# Autodesk Inventor assembly: Lady Brown
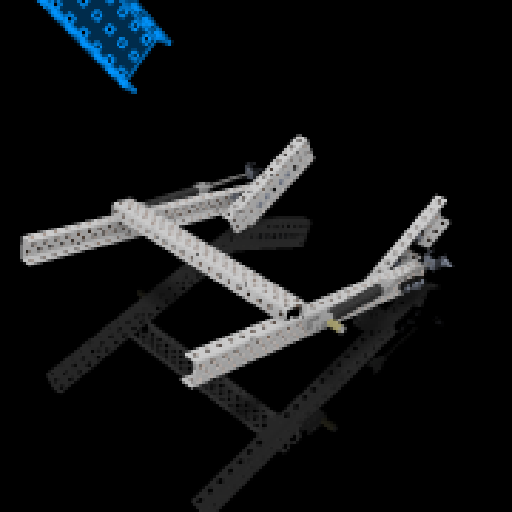
[picture p0: Inventor's stored thumbnail of the model, 512x512]
Saved by Autodesk Inventor 2025 (Build 290162000, 162)
## iProperties
Created: 2024-12-19
Part Number: Lady Brown
Document SubType Name: Assembly
Designer: Juan
Author: Juan
## Documents named in this file (20)
- C:\Users\Juan\Documents\GitHub\ATUM-VRC-High-Stakes-CAD\Robot\Subassemblies\Lady Brown.iam
- C:\Users\Juan\Documents\GitHub\ATUM-VRC-High-Stakes-CAD\VEX-CAD-Inventor\Structure\C Channel\Aluminum 1x2x1\Alu C 1x2x1x25.ipt
- C:\Users\Juan\Documents\GitHub\ATUM-VRC-High-Stakes-CAD\VEX-CAD-Inventor\Structure\C Channel\Aluminum 1x2x1\Alu C 1x2x1x19.ipt
- C:\Users\Juan\Documents\GitHub\ATUM-VRC-High-Stakes-CAD\VEX-CAD-Inventor\Motion\Spacers\Spacer Nylon .375 OD\NSpacer .375 OD x .500.ipt
- C:\Users\Juan\Documents\GitHub\ATUM-VRC-High-Stakes-CAD\VEX-CAD-Inventor\Motion\Spacers\Spacer Nylon .375 OD.ipt
- C:\Users\Juan\Documents\GitHub\ATUM-VRC-High-Stakes-CAD\VEX-CAD-Inventor\Motion\Pneumatics\Reference Parts\Pistons\Double Acting Piston Body.ipt
- C:\Users\Juan\Documents\GitHub\ATUM-VRC-High-Stakes-CAD\VEX-CAD-Inventor\Motion\Pneumatics\Reference Parts\Pistons\Double Acting Piston Rod.ipt
- C:\Users\Juan\Documents\GitHub\ATUM-VRC-High-Stakes-CAD\VEX-CAD-Inventor\Motion\Pneumatics\Legacy - SMC Pneumatics\Fitting for Cylinders.ipt
- C:\Users\Juan\Documents\GitHub\ATUM-VRC-High-Stakes-CAD\VEX-CAD-Inventor\Motion\Shaft LS\Bearing Flat.ipt
- C:\Users\Juan\Documents\GitHub\ATUM-VRC-High-Stakes-CAD\VEX-CAD-Inventor\Structure\Hardware\Screw Steel - Star\SScrew Star Smooth .500.ipt
- C:\Users\Juan\Documents\GitHub\ATUM-VRC-High-Stakes-CAD\VEX-CAD-Inventor\Structure\Hardware\Screw Steel - Star.ipt
- C:\Users\Juan\Documents\GitHub\ATUM-VRC-High-Stakes-CAD\VEX-CAD-Inventor\Structure\C Channel\Aluminum 1x3x1\Alu C 1x3x1x11.ipt
- C:\Users\Juan\Documents\GitHub\ATUM-VRC-High-Stakes-CAD\VEX-CAD-Inventor\Motion\1-Post Bearing Flat Hex Retainer.ipt
- C:\Users\Juan\Documents\GitHub\ATUM-VRC-High-Stakes-CAD\VEX-CAD-Inventor\Motion\Pneumatics\Legacy - SMC Pneumatics\Cylinder Mount.ipt
- C:\Users\Juan\Documents\GitHub\ATUM-VRC-High-Stakes-CAD\VEX-CAD-Inventor\Motion\Spacers\Spacer Nylon .375 OD\NSpacer .375 OD x .375.ipt
- C:\Users\Juan\Documents\GitHub\ATUM-VRC-High-Stakes-CAD\VEX-CAD-Inventor\Structure\Hardware\Screw Steel - Star\SScrew Star Smooth 2.250.ipt
- C:\Users\Juan\Documents\GitHub\ATUM-VRC-High-Stakes-CAD\VEX-CAD-Inventor\Structure\Hardware\Nut Nylock.ipt
- C:\Users\Juan\Documents\GitHub\ATUM-VRC-High-Stakes-CAD\VEX-CAD-Inventor\Structure\Hardware\Screw Steel - Star\SScrew Star Smooth 1.750.ipt
- C:\Users\Juan\Documents\GitHub\ATUM-VRC-High-Stakes-CAD\VEX-CAD-Inventor\Structure\Hardware\Nut Thin Nylock.ipt
- C:\Users\Juan\Documents\GitHub\ATUM-VRC-High-Stakes-CAD\VEX-CAD-Inventor\Structure\Hardware\Screw Steel - Star\SScrew Star Smooth .375.ipt
## Components (57 placed, 17 different names)
1. Alu C 1x2x1x25:1
2. Alu C 1x2x1x25:2
3. Alu C 1x2x1x19:1
4. NSpacer .375 OD x .500:1
5. NSpacer .375 OD x .500:2
6. Double Acting Piston Body:1
7. Double Acting Piston Rod:1
8. Fitting for Cylinders:1
9. Bearing Flat:1
10. SScrew Star Smooth .500:1
11. SScrew Star Smooth .500:2
12. Alu C 1x3x1x11:1
13. 1-Post Bearing Flat Hex Retainer:1
14. 1-Post Bearing Flat Hex Retainer:2
15. Cylinder Mount:1
16. NSpacer .375 OD x .375:3
17. NSpacer .375 OD x .500:4
18. NSpacer .375 OD x .375:5
19. NSpacer .375 OD x .500:6
20. SScrew Star Smooth 2.250:3
21. Nut Nylock:1
22. SScrew Star Smooth 1.750:4
23. Nut Thin Nylock:1
24. Nut Nylock:2
25. SScrew Star Smooth .375:5
26. SScrew Star Smooth .375:6
27. Nut Nylock:3
28. Double Acting Piston Body:2
29. Double Acting Piston Rod:2
30. NSpacer .375 OD x .500:13
31. NSpacer .375 OD x .375:14
32. Nut Thin Nylock:4
33. Nut Thin Nylock:3
34. Nut Thin Nylock:6
35. Nut Thin Nylock:5
36. SScrew Star Smooth 2.250:12
37. NSpacer .375 OD x .500:12
38. Fitting for Cylinders:2
39. Bearing Flat:2
40. SScrew Star Smooth .500:7
41. SScrew Star Smooth .500:8
42. Alu C 1x3x1x11:2
43. NSpacer .375 OD x .500:10
44. NSpacer .375 OD x .500:11
45. Cylinder Mount:2
46. NSpacer .375 OD x .500:7
47. Nut Nylock:4
48. Nut Thin Nylock:2
49. Nut Nylock:5
50. SScrew Star Smooth .375:9
51. SScrew Star Smooth .375:10
52. Nut Nylock:6
53. 1-Post Bearing Flat Hex Retainer:3
54. 1-Post Bearing Flat Hex Retainer:4
55. SScrew Star Smooth 1.750:11
56. NSpacer .375 OD x .500:8
57. NSpacer .375 OD x .375:9
## Relationships (93: Mate 58, WeldJoint 32, CylindricalJoint 2, RevoluteJoint 1)
- [Mate]: Alu C 1x2x1x25:1 ↔ Alu C 1x2x1x19:1
- [Mate]: Alu C 1x2x1x25:1 ↔ Alu C 1x2x1x19:1
- [Mate]: Alu C 1x2x1x25:2 ↔ Alu C 1x2x1x19:1
- [Mate]: Alu C 1x2x1x25:2 ↔ Alu C 1x2x1x19:1
- [Mate]: Alu C 1x2x1x19:1 ↔ NSpacer .375 OD x .500:1
- [Mate]: Alu C 1x2x1x19:1 ↔ NSpacer .375 OD x .500:2
- [Mate]: Alu C 1x2x1x19:1 ↔ NSpacer .375 OD x .500:2
- [Mate]: Alu C 1x2x1x19:1 ↔ NSpacer .375 OD x .500:1
- [Mate]: Alu C 1x2x1x25:1 ↔ NSpacer .375 OD x .500:2
- [Mate]: Double Acting Piston Body:1 ↔ Double Acting Piston Rod:1
- [CylindricalJoint]: Double Acting Piston Body:1 ↔ Double Acting Piston Rod:1
- [Mate]: Double Acting Piston Body:1 ↔ Fitting for Cylinders:1
- [Mate]: Double Acting Piston Body:1 ↔ Fitting for Cylinders:1
- [Mate]: Alu C 1x2x1x25:1 ↔ Bearing Flat:1
- [Mate]: Alu C 1x2x1x25:1 ↔ Bearing Flat:1
- [Mate]: Alu C 1x2x1x25:1 ↔ Bearing Flat:1
- [WeldJoint]: Bearing Flat:1 ↔ SScrew Star Smooth .500:2
- [WeldJoint]: Bearing Flat:1 ↔ SScrew Star Smooth .500:1
- [Mate]: Alu C 1x3x1x11:1 ↔ 1-Post Bearing Flat Hex Retainer:2
- [Mate]: Alu C 1x3x1x11:1 ↔ 1-Post Bearing Flat Hex Retainer:2
- [Mate]: Alu C 1x3x1x11:1 ↔ 1-Post Bearing Flat Hex Retainer:1
- [Mate]: Alu C 1x3x1x11:1 ↔ 1-Post Bearing Flat Hex Retainer:1
- [Mate]: Alu C 1x3x1x11:1 ↔ 1-Post Bearing Flat Hex Retainer:2
- [Mate]: Alu C 1x3x1x11:1 ↔ 1-Post Bearing Flat Hex Retainer:1
- [Mate]: Bearing Flat:1 ↔ 1-Post Bearing Flat Hex Retainer:2
- [Mate]: Double Acting Piston Rod:1 ↔ Cylinder Mount:1
- [Mate]: 1-Post Bearing Flat Hex Retainer:1 ↔ Cylinder Mount:1
- [WeldJoint]: NSpacer .375 OD x .500:4 ↔ NSpacer .375 OD x .375:5
- [Mate]: Cylinder Mount:1 ↔ NSpacer .375 OD x .500:6
- [Mate]: Cylinder Mount:1 ↔ NSpacer .375 OD x .500:6
- [WeldJoint]: Alu C 1x3x1x11:1 ↔ SScrew Star Smooth 2.250:3
- [WeldJoint]: Cylinder Mount:1 ↔ Nut Nylock:1
- [WeldJoint]: Alu C 1x3x1x11:1 ↔ SScrew Star Smooth 1.750:4
- [WeldJoint]: Bearing Flat:1 ↔ Nut Thin Nylock:1
- [WeldJoint]: Alu C 1x3x1x11:1 ↔ SScrew Star Smooth .375:6
- [WeldJoint]: Alu C 1x3x1x11:1 ↔ SScrew Star Smooth .375:5
- [WeldJoint]: 1-Post Bearing Flat Hex Retainer:1 ↔ Nut Nylock:2
- [WeldJoint]: 1-Post Bearing Flat Hex Retainer:2 ↔ Nut Nylock:3
- [Mate]: Double Acting Piston Body:2 ↔ Double Acting Piston Rod:2
- [Mate]: Double Acting Piston Body:2 ↔ Fitting for Cylinders:2
- [Mate]: Double Acting Piston Body:2 ↔ Fitting for Cylinders:2
- [Mate]: Double Acting Piston Rod:2 ↔ Cylinder Mount:2
- [Mate]: Cylinder Mount:2 ↔ NSpacer .375 OD x .500:7
- [CylindricalJoint]: Double Acting Piston Body:2 ↔ Double Acting Piston Rod:2
- [WeldJoint]: Bearing Flat:2 ↔ SScrew Star Smooth .500:7
- [WeldJoint]: Bearing Flat:2 ↔ SScrew Star Smooth .500:8
- [WeldJoint]: Cylinder Mount:2 ↔ Nut Nylock:4
- [WeldJoint]: Bearing Flat:2 ↔ Nut Thin Nylock:2
- [WeldJoint]: Alu C 1x3x1x11:2 ↔ SScrew Star Smooth .375:9
- [WeldJoint]: Alu C 1x3x1x11:2 ↔ SScrew Star Smooth .375:10
- [Mate]: Alu C 1x3x1x11:2 ↔ 1-Post Bearing Flat Hex Retainer:3
- [Mate]: Alu C 1x3x1x11:2 ↔ 1-Post Bearing Flat Hex Retainer:3
- [Mate]: Alu C 1x3x1x11:2 ↔ 1-Post Bearing Flat Hex Retainer:3
- [Mate]: Alu C 1x3x1x11:2 ↔ 1-Post Bearing Flat Hex Retainer:4
- [Mate]: Alu C 1x3x1x11:2 ↔ 1-Post Bearing Flat Hex Retainer:4
- [Mate]: Alu C 1x3x1x11:2 ↔ 1-Post Bearing Flat Hex Retainer:4
- [WeldJoint]: Alu C 1x3x1x11:2 ↔ SScrew Star Smooth 1.750:11
- [Mate]: Alu C 1x2x1x25:2 ↔ Bearing Flat:2
- [Mate]: Alu C 1x2x1x25:2 ↔ Bearing Flat:2
- [Mate]: Alu C 1x2x1x25:2 ↔ Bearing Flat:2
- [Mate]: Bearing Flat:2 ↔ SScrew Star Smooth 1.750:11
- [Mate]: Cylinder Mount:2 ↔ NSpacer .375 OD x .500:7
- [WeldJoint]: Nut Nylock:5 ↔ 1-Post Bearing Flat Hex Retainer:3
- [WeldJoint]: Nut Nylock:6 ↔ 1-Post Bearing Flat Hex Retainer:4
- [WeldJoint]: NSpacer .375 OD x .500:8 ↔ NSpacer .375 OD x .375:9
- [Mate]: Alu C 1x2x1x25:2 ↔ Double Acting Piston Body:2
- [Mate] (0.7937 mm): Alu C 1x2x1x25:2 ↔ Double Acting Piston Body:2
- [Mate]: Alu C 1x3x1x11:1 ↔ Alu C 1x3x1x11:2
- [Mate]: Alu C 1x3x1x11:1 ↔ Alu C 1x3x1x11:2
- [RevoluteJoint] (0.7937 mm): Alu C 1x2x1x25:1 ↔ Double Acting Piston Body:1
- [WeldJoint] (6.35 mm): Double Acting Piston Rod:1 ↔ Cylinder Mount:1
- [WeldJoint] (6.35 mm): Double Acting Piston Rod:2 ↔ Cylinder Mount:2
- [Mate]: Cylinder Mount:2 ↔ NSpacer .375 OD x .375:9
- [Mate]: 1-Post Bearing Flat Hex Retainer:2 ↔ NSpacer .375 OD x .375:3
- [WeldJoint]: Cylinder Mount:1 ↔ NSpacer .375 OD x .375:5
- [Mate]: Alu C 1x2x1x25:2 ↔ NSpacer .375 OD x .500:11
- [Mate]: Alu C 1x2x1x25:2 ↔ NSpacer .375 OD x .500:10
- [Mate]: Alu C 1x2x1x25:2 ↔ NSpacer .375 OD x .500:10
- [Mate]: Alu C 1x2x1x25:2 ↔ NSpacer .375 OD x .500:11
- [Mate]: Alu C 1x2x1x19:1 ↔ NSpacer .375 OD x .500:11
- [WeldJoint]: Alu C 1x2x1x25:1 ↔ NSpacer .375 OD x .500:12
- [WeldJoint]: NSpacer .375 OD x .375:3 ↔ NSpacer .375 OD x .500:12
- [WeldJoint]: NSpacer .375 OD x .500:13 ↔ NSpacer .375 OD x .375:14
- [Mate]: NSpacer .375 OD x .500:13 ↔ SScrew Star Smooth 1.750:11
- [Mate]: Alu C 1x2x1x25:2 ↔ NSpacer .375 OD x .500:13
- [Mate]: NSpacer .375 OD x .375:14 ↔ 1-Post Bearing Flat Hex Retainer:4
- [WeldJoint]: Alu C 1x2x1x25:1 ↔ Nut Thin Nylock:4
- [WeldJoint]: Alu C 1x2x1x25:1 ↔ Nut Thin Nylock:3
- [WeldJoint]: SScrew Star Smooth 2.250:12 ↔ Alu C 1x3x1x11:2
- [WeldJoint]: Alu C 1x2x1x25:2 ↔ Nut Thin Nylock:6
- [WeldJoint]: Alu C 1x2x1x25:2 ↔ Nut Thin Nylock:5
- [Mate]: SScrew Star Smooth 2.250:12 ↔ Nut Nylock:4
- [Mate]: SScrew Star Smooth 2.250:12 ↔ NSpacer .375 OD x .375:9
## Named parameters: d1821_d1818 = 0 mm, d1789_d1094 = 0 mm, d1790_d1097 = 0 mm, d1791_d1068_d1063 = 0 mm, d1792_d1069_d1064 = 0 deg, d1793_d1070_d1065 = -19.05 mm, d1794_d1071_d1066 = -69.85 mm, d1795_d1072_d1067 = -69.85 mm
